# Autodesk Inventor assembly: HSR35R1SS-280L_G20_0_B-M6F_85-3_0_0_0_1_(R2)
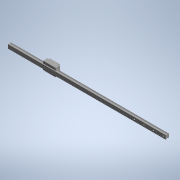
[picture p0: Inventor's stored thumbnail of the model, 180x180]
Saved by Autodesk Inventor 2022 (Build 260153000, 153)
## iProperties
Category: PARTsolutions
Company: THK
Part Number: HSR35R1SS-280L_G20_0_B-M6F_85-3_0_0_0_1_(R2)
Catalog Web Link: www.cadenas.de
Description: Compact Type - Heavy Load HSR-R-
Vendor: THK
Document SubType Name: Assembly
Designer: partserver
Manufacturer: THK
Mass: 483.854 g
Surface Area: 788.239 cm^2
Volume: 483.854 cm^3
Density: 1 g/cm^3
PSOL_IDENT_0: {$CADENAS_DATA\23d-libs\thk\linear_motion_systems\lm_guide\lm_guide\lm_guide_hsr\four_taped_hole_typ
PSOL_IDENT_1: e\hsr_r_asmtab.prj},334 {VTYP=3D},{STYP=ASSTAB},{NB=HSR35R1SS-280L_G20_0_B-M6F_85-3_0_0_0_1_(R2)},{L
PSOL_IDENT_2: INA=HSR35R1SS+280L (G20g20, B-M6F)},{NN=Compact Type - Heavy Load HSR-R},{DATE=21.06.2021 00:23:41},
PSOL_IDENT_3: {GEOMDATE=24.03.2021 07:03:45},{VERSION=},{LINEID=70},{WBVAR=NOB,QZ,SO,RADC,L,ACCG,G,GX,NR,POR,GPJ,T
PSOL_IDENT_4: APH,P1,P2,P3,P4,TH},{WBNUMERIC=NOB,L,GX,POR,P1,P2,P3,P4}  {NB=HSR35R1SS-280L_G20_0_B-M6F_85-3_0_0_0_
PSOL_IDENT_5: 1_(R2)},{LINA=HSR35R1SS+280L (G20g20, B-M6F)},{KT=DUMMY},{MN=HSR35R},{PD=280},{NOB=1},{QZ=},{SO=SS},
PSOL_IDENT_6: {RADC=},{L=280.0},{ACCG=},{L1=80.40},{L3=11.000},{L4=1.5},{L5=2},{G=},{INFO=Infotext},{SO1='SS','SS-
PSOL_IDENT_7: With end, side seals','','Without Seals','UU','UU- With end seals (on both ends)','DD','DD- With do
PSOL_IDENT_8: uble, side, inner seals','ZZ','ZZ- With end, side, inner seals and metal scrapers','KK','KK- With do
PSOL_IDENT_9: uble, side, inner seals and metal scrapers','SSHH','SSHH- With end, side, inner seals and LaCS','DDH
PSOL_IDENT_10: H','DDHH- With double, side, inner seals and LaCS','ZZHH','ZZHH- With end, side, inner seals and met
PSOL_IDENT_11: al scrapers and LaCS','KKHH','KKHH- With double, side, inner seals and metal scrapers and LaCS'},{LX=
PSOL_IDENT_12: 109.4},{EX=11.6},{LLL=121},{L0=121},{LMIN=122.0},{LMINX=122.0},{GG='', 'Symmetrical (G1=G2)', 'A', '
PSOL_IDENT_13: Asymmetrical'},{GX=20},{GX2=20.00},{GX1=20},{NOTE=},{RC1=No connection},{NR=},{POR=0},{POR1=0,[0:0]}
PSOL_IDENT_14: ,{GPJ=B-M6F},{TAPH=},{INFO1=Infotext},{P1=85.3},{P2=0},{P3=0},{P4=0},{TH=1},{LEND=8640.00},{LPORM=80
PSOL_IDENT_15: .00},{LPORX=1000.00},{GPJ1=<'B-M6F','B-M6F'>,'', 'None', 'A-M6F','A-M6F','C-M6F','C-M6F', 'LF-A','LF
PSOL_IDENT_16: -A','LF-B','LF-B', 'SF-A','SF-A','SF-B','SF-B'},{PSM1=0},{PSM2=0},{PSM3=0},{PSM4=0},{PS1=170.6},{PS2=
PSOL_IDENT_17: 0},{PS3=0},{PS4=0},{PSX2=0},{PSX3=0},{PSX4=0},{LTR=109.40},{F=80.00},{D1=9.00},{D2=14.00},{HM=12.00}
PSOL_IDENT_18: ,{MAXL=3000.00},{GMIN=8},{GMX=20},{GMAX1=3.3},{G1=14},{G2=14},{NX=1},{LT=2880.00},{A=4},{LF=294},{LM=
PSOL_IDENT_19: 280},{LL=266},{AA=3},{GA=20.00},{GMAX=32},{RCX=},{H3=7.50},{ND=5.000},{ON=HSR35R},{ON1=},{NRR=},{QZX=''
PSOL_IDENT_20: ,'No','QZ','Yes'},{LP=2},{NRX=},{INFOX=block1_1_},{PPATH=hsr_r/hsr_r_asmtpl.prj},{GPJX=2},{QZZ=},{IN
PSOL_IDENT_21: FOX2=dim_},{PD1=85.3},{LMIN11=280.0},{TX=},{GPJE=},{ND100=35},{GPJNB=_B-M6F},{GNB=},{LINT=280},{LTEX
PSOL_IDENT_22: T=280},{LREST=},{LNB=280},{GXINT=20},{GXTEXT=20},{GXREST=},{GXNB=20},{PORINT=0},{PORTEXT=0},{PORREST=
PSOL_IDENT_23: },{PORNB=0},{P1INT=85},{P1TEXT=85.3},{P1REST=3},{P1NB=85-3},{P2INT=0},{P2TEXT=0},{P2REST=},{P2NB=0},
PSOL_IDENT_24: {P3INT=0},{P3TEXT=0},{P3REST=},{P3NB=0},{P4INT=0},{P4TEXT=0},{P4REST=},{P4NB=0},{ORDERNONB=HSR35R1SS
PSOL_IDENT_25: -280L},{CNSORDERNO=HSR35R1SS_B-M6F+280L-R2},{REV=R2},{X=1},{NOTE2=If you hope to avoid collision bet
PSOL_IDENT_26: ween LM block mounting hole and the mounting bolt, select \"Nominal diameter of the female screw\" w
PSOL_IDENT_27: ith the above selection.},{RADCX='','No Symbol : Normal','C1','C1 : Light preload','C0','C0 : Medium
PSOL_IDENT_28: preload'},{ACCGX='','No Symbol : Normal grade','H','H : High-accuracy grade','P','P : Precision gra
PSOL_IDENT_29: de','SP','SP : Super precision grade','UP','UP : Ultra precision grade'},{CNSORDERNO2=HSR35R1SS+280L
PSOL_IDENT_30: (G20g20, B-M6F)},{TAPHX='', 'No', 'K', 'Yes'},{TYPECODE=HSR35R1SS+280L}
NB: HSR35R1SS-280L_G20_0_B-M6F_85-3_0_0_0_1_(R2)
NN: Compact Type - Heavy Load HSR-R
NBSYN: $ORDERNONB.$GNB._G$GXNB._$PORNB.$GPJNB._$P1NB._$P2NB._$P3NB._$P4NB._$TH._$TAPH.($REV.)
LINA: HSR35R1SS+280L (G20g20, B-M6F)
CATALOG: THK
MN: HSR35R
NOB: 1
QZ: No
SO: SS- With end, side seals
RADC: No Symbol : Normal
L: 280
ACCG: No Symbol : Normal grade
G: Symmetrical (G1=G2)
INFO: Infotext
GX: 20
GX2: 20
RC1: No connection
POR: 0
GPJ: B-M6F
TAPH: No
INFO1: Infotext
P1: 85.3
P2: 0
P3: 0
P4: 0
TH: Minor diameter of thread
NOTE2: If you hope to avoid collision between LM block mounting hole and the mounting bolt, select "Nominal diameter of the female screw" with the above selection.
SUPPLIER: THK
ARTICLENO: HSR35R1SS-280L_G20_0_B-M6F_85-3_0_0_0_1_(R2)
BOMINFO: HSR35R1SS+280L (G20g20, B-M6F)
CREATOR: CADENAS GmbH
Title: HSR35R1SS+280L (G20g20, B-M6F)
Author: Cadenas PARTsolutions
## Documents named in this file (4)
- \\Mac\Home\Desktop\WinnipegPMTTestFacility\gantry design\THK_HSR35R1SS280LG200BM6F8530001R20\AIS2020\HSR35R1SS-280L_G20_0_B-M6F_85-3_0_0_0_1_(R2).iam
- \\Mac\Home\Desktop\WinnipegPMTTestFacility\gantry design\THK_HSR35R1SS280LG200BM6F8530001R20\AIS2020\HSR35R128020 Rail.ipt
- \\Mac\Home\Desktop\WinnipegPMTTestFacility\gantry design\THK_HSR35R1SS280LG200BM6F8530001R20\AIS2020\HSR35RSSB-M6F1 Slider-1-R2.ipt
- \\Mac\Home\Desktop\WinnipegPMTTestFacility\gantry design\THK_HSR35R1SS280LG200BM6F8530001R20\AIS2020\hsr_ftht_B-M6F_grease_nipple_joint.ipt
## Components (3 placed, 3 different names)
1. HSR35R128020 Rail:1
2. HSR35RSSB-M6F1 Slider-1-R2:1
3. hsr_ftht_B-M6F_grease_nipple_joint:1
## Relationships (1: Flush 1)
- Flush:1 (457.2 mm)
